# Autodesk Inventor assembly: Weapon Assembly
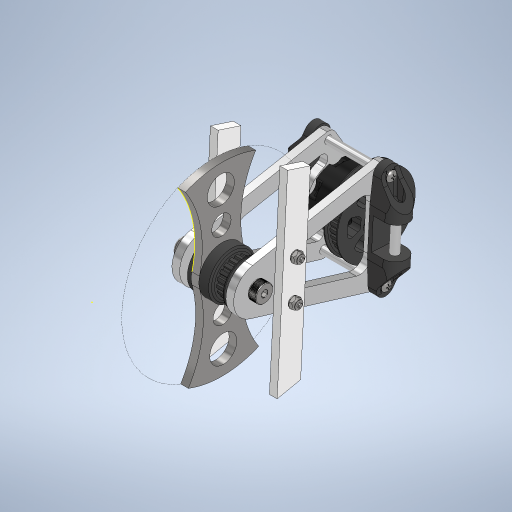
[picture p0: Inventor's stored thumbnail of the model, 512x512]
Saved by Autodesk Inventor 2023.1 (Build 271208000, 208)
## iProperties
Created: 2022-05-21
Part Number: Weapon Assembly
Document SubType Name: Assembly
Designer: Nathan Cai
Mass: 716.023 g
Surface Area: 1380.74 cm^2
Volume: 212.806 cm^3
Density: 3.36467 g/cm^3
Author: Nathan Cai
## Documents named in this file (15)
- E:\Documents\Inventor\0.3rd Lawette - V3.4\Vertical Weapon Assembly (Type A)\Weapon Assembly (Vert A).iam
- E:\Documents\Inventor\0.3rd Lawette - V3.4\Vertical Weapon Assembly (Type A)\Weapon (Weapon-Side Pulley).iam
- E:\Documents\Inventor\0.3rd Lawette - V3.4\Vertical Weapon Assembly (Type A)\90807A139_Same-Size Thread Alloy Steel Shoulder Screw.ipt
- E:\Documents\Inventor\0.3rd Lawette - V3.4\Vertical Weapon Assembly (Type A)\90630A121_High-Strength Steel Nylon-Insert Locknut.ipt
- E:\Documents\Inventor\0.3rd Lawette - V3.4\Vertical Weapon Assembly (Type A)\Weapon (Motor-Side Pulley).iam
- E:\Documents\Inventor\0.3rd Lawette - V3.4\Vertical Weapon Assembly (Type A)\Frame (Clear Side).ipt
- E:\Documents\Inventor\0.3rd Lawette - V3.4\Standoff 1.5in.ipt
- E:\Documents\Inventor\0.3rd Lawette - V3.4\Vertical Weapon Assembly (Type A)\Legs.ipt
- E:\Documents\Inventor\Content Center Files\R2023\en-US\ANSI B18.6.3(27)\ANSI B18.6.3 - 6-32 UNC - 0.75(11).ipt
- E:\Documents\Inventor\Content Center Files\R2023\en-US\SAE J773b\SAE J773b - No. 6. SAE Type L. narrow.ipt
- E:\Documents\Inventor\Content Center Files\R2023\en-US\IFI 100 107(2)\IFI 100_107 - No. 6 - 32 Metal Type.ipt
- E:\Documents\Inventor\0.3rd Lawette - V3.4\Vertical Weapon Assembly (Type A)\Frame (Motor Side).ipt
- E:\Documents\Inventor\0.3rd Lawette - V3.4\Vertical Weapon Assembly (Type A)\Legs_MIR.ipt
- E:\Documents\Inventor\0.3rd Lawette - V3.4\Bracket.ipt
- E:\Documents\Inventor\Content Center Files\R2023\en-US\ANSI B18.6.3(27)\ANSI B18.6.3 - 6-32 UNC - 0.625(11).ipt
## Components (42 placed, 14 different names)
1. Weapon (Weapon-Side Pulley):1 [sub-assembly] — Mate:3
2. Weapon (Motor-Side Pulley):1 [sub-assembly] — Mate:167, Mate:168, Mate:169
3. 90807A139_Same-Size Thread Alloy Steel Shoulder Screw:1 — Mate:1, Mate:2, Mate:3, Mate:9, Mate:10
4. 90630A121_High-Strength Steel Nylon-Insert Locknut:1 — Mate:1, Mate:2
5. Frame (Motor Side):1 — Symmetry:1, Mate:146, Mate:147, Mate:148, Mate:151, Mate:152, Mate:153, Mate:154, Mate:155, Mate:157, Mate:167, Mate:168, Mate:169, Mate:170
6. Frame (Clear Side):1 — Mate:9, Mate:10, Mate:28, Mate:29, Mate:30, Mate:102, Symmetry:1, Mate:159, Mate:160, Mate:161, Mate:162, Mate:163, Mate:165, Mate:173
7. Legs:1 — Mate:28, Mate:29, Mate:30, Mate:164, Mate:166
8. Legs_MIR:1 — Mate:146, Mate:147, Mate:148, Mate:156, Mate:158
9. Bracket:1 — Mate:173, Mate:174, Mate:175, Mate:176, Flush:2, Mate:178, Mate:179, Mate:180, Mate:181, Mate:186, Mate:187, Mate:189, Mate:190
10. Bracket:2 — Mate:170, Mate:171, Mate:172, Mate:177, Flush:1, Mate:182, Mate:183, Mate:184, Mate:185, Mate:188, Mate:192
11. Standoff 1.5in:1 — Mate:102, Mate:171, Mate:174
12. Standoff 1.5in:2 — Mate:172, Mate:175
13. Standoff 1.5in:3 — Mate:176, Flush:2, Mate:191, Mate:193
14. Standoff 1.5in:4 — Mate:177, Flush:1
15. Cross Recessed Truss Head Machine Screw - Type I - Inch No. 6 - 32 - 3/4:8 — Mate:151, Mate:152
16. Conical Spring Washer SAE J773b (Inch) No. 6. SAE Type L. narrow:11 — Mate:155, Mate:156, Insert:21
17. Prevailing Torque Type Hex Nut - Inch (IFI) No. 6 - 32 Metal Type:11 — Insert:21
18. Cross Recessed Truss Head Machine Screw - Type I - Inch No. 6 - 32 - 3/4:10 — Mate:159, Mate:160
19. Conical Spring Washer SAE J773b (Inch) No. 6. SAE Type L. narrow:13 — Mate:163, Mate:164, Insert:23
20. Prevailing Torque Type Hex Nut - Inch (IFI) No. 6 - 32 Metal Type:13 — Insert:23
21. Cross Recessed Truss Head Machine Screw - Type I - Inch No. 6 - 32 - 3/4:14 — Mate:153, Mate:154
22. Conical Spring Washer SAE J773b (Inch) No. 6. SAE Type L. narrow:17 — Mate:157, Mate:158, Insert:22
23. Prevailing Torque Type Hex Nut - Inch (IFI) No. 6 - 32 Metal Type:17 — Insert:22
24. Cross Recessed Truss Head Machine Screw - Type I - Inch No. 6 - 32 - 3/4:15 — Mate:161, Mate:162
25. Conical Spring Washer SAE J773b (Inch) No. 6. SAE Type L. narrow:18 — Mate:165, Mate:166, Insert:24
26. Prevailing Torque Type Hex Nut - Inch (IFI) No. 6 - 32 Metal Type:18 — Insert:24
27. Conical Spring Washer SAE J773b (Inch) No. 6. SAE Type L. narrow:19 — Mate:178, Mate:179, Insert:25
28. Cross Recessed Truss Head Machine Screw - Type I - Inch No. 6 - 32 - 3/4:16 — Insert:25
29. Conical Spring Washer SAE J773b (Inch) No. 6. SAE Type L. narrow:20 — Mate:180, Mate:181, Insert:26
30. Cross Recessed Truss Head Machine Screw - Type I - Inch No. 6 - 32 - 3/4:17 — Insert:26
31. Conical Spring Washer SAE J773b (Inch) No. 6. SAE Type L. narrow:21 — Mate:182, Mate:183, Insert:27
32. Cross Recessed Truss Head Machine Screw - Type I - Inch No. 6 - 32 - 3/4:18 — Insert:27
33. Conical Spring Washer SAE J773b (Inch) No. 6. SAE Type L. narrow:22 — Mate:184, Mate:185, Insert:28
34. Cross Recessed Truss Head Machine Screw - Type I - Inch No. 6 - 32 - 3/4:19 — Insert:28
35. Conical Spring Washer SAE J773b (Inch) No. 6. SAE Type L. narrow:23 — Mate:186, Mate:187, Insert:29
36. Cross Recessed Truss Head Machine Screw - Type I - Inch No. 6 - 32 - 5/8:1 — Insert:29
37. Conical Spring Washer SAE J773b (Inch) No. 6. SAE Type L. narrow:24 — Mate:188, Mate:189, Insert:30
38. Cross Recessed Truss Head Machine Screw - Type I - Inch No. 6 - 32 - 5/8:2 — Insert:30
39. Conical Spring Washer SAE J773b (Inch) No. 6. SAE Type L. narrow:25 — Mate:190, Mate:191, Insert:31
40. Cross Recessed Truss Head Machine Screw - Type I - Inch No. 6 - 32 - 5/8:3 — Insert:31
41. Conical Spring Washer SAE J773b (Inch) No. 6. SAE Type L. narrow:26 — Mate:192, Mate:193, Insert:32
42. Cross Recessed Truss Head Machine Screw - Type I - Inch No. 6 - 32 - 5/8:4 — Insert:32
## Relationships (77: Mate 62, Insert 12, Flush 2, Symmetry 1)
- Mate:1: 90807A139_Same-Size Thread Alloy Steel Shoulder Screw:1 ↔ 90630A121_High-Strength Steel Nylon-Insert Locknut:1
- Mate:2 (50.8 mm): 90807A139_Same-Size Thread Alloy Steel Shoulder Screw:1 ↔ 90630A121_High-Strength Steel Nylon-Insert Locknut:1
- Mate:3: Weapon (Weapon-Side Pulley):1 ↔ 90807A139_Same-Size Thread Alloy Steel Shoulder Screw:1
- [Mate]: 90807A139_Same-Size Thread Alloy Steel Shoulder Screw:1 ↔ Frame (Motor Side):1
- Mate:9: 90807A139_Same-Size Thread Alloy Steel Shoulder Screw:1 ↔ Frame (Clear Side):1
- Mate:10: 90807A139_Same-Size Thread Alloy Steel Shoulder Screw:1 ↔ Frame (Clear Side):1
- [Mate]: Frame (Motor Side):1 ↔ Frame (Clear Side):1
- [Mate]: Frame (Motor Side):1 ↔ Standoff 1.5in:1
- [Mate]: Frame (Motor Side):1 ↔ Standoff 1.5in:2
- [Mate]: Frame (Motor Side):1 ↔ Standoff 1.5in:1
- [Mate]: Frame (Motor Side):1 ↔ Standoff 1.5in:2
- Mate:28: Frame (Clear Side):1 ↔ Legs:1
- Mate:29: Frame (Clear Side):1 ↔ Legs:1
- Mate:30: Frame (Clear Side):1 ↔ Legs:1
- Mate:102: Frame (Clear Side):1 ↔ Standoff 1.5in:1
- [Mate] (0.0254 mm): Weapon (Weapon-Side Pulley):1 ↔ Frame (Motor Side):1
- Symmetry:1: Frame (Motor Side):1 ↔ Frame (Clear Side):1
- Mate:146: Frame (Motor Side):1 ↔ Legs_MIR:1
- Mate:147: Frame (Motor Side):1 ↔ Legs_MIR:1
- Mate:148: Frame (Motor Side):1 ↔ Legs_MIR:1
- Mate:151: Frame (Motor Side):1 ↔ Cross Recessed Truss Head Machine Screw - Type I - Inch No. 6 - 32 - 3/4:8
- Mate:152: Frame (Motor Side):1 ↔ Cross Recessed Truss Head Machine Screw - Type I - Inch No. 6 - 32 - 3/4:8
- Mate:153: Frame (Motor Side):1 ↔ Cross Recessed Truss Head Machine Screw - Type I - Inch No. 6 - 32 - 3/4:14
- Mate:154: Frame (Motor Side):1 ↔ Cross Recessed Truss Head Machine Screw - Type I - Inch No. 6 - 32 - 3/4:14
- Mate:155: Frame (Motor Side):1 ↔ Conical Spring Washer SAE J773b (Inch) No. 6. SAE Type L. narrow:11
- Mate:156: Legs_MIR:1 ↔ Conical Spring Washer SAE J773b (Inch) No. 6. SAE Type L. narrow:11
- Mate:157: Frame (Motor Side):1 ↔ Conical Spring Washer SAE J773b (Inch) No. 6. SAE Type L. narrow:17
- Mate:158: Legs_MIR:1 ↔ Conical Spring Washer SAE J773b (Inch) No. 6. SAE Type L. narrow:17
- Insert:21: Conical Spring Washer SAE J773b (Inch) No. 6. SAE Type L. narrow:11 ↔ Prevailing Torque Type Hex Nut - Inch (IFI) No. 6 - 32 Metal Type:11
- Insert:22: Conical Spring Washer SAE J773b (Inch) No. 6. SAE Type L. narrow:17 ↔ Prevailing Torque Type Hex Nut - Inch (IFI) No. 6 - 32 Metal Type:17
- Mate:159: Frame (Clear Side):1 ↔ Cross Recessed Truss Head Machine Screw - Type I - Inch No. 6 - 32 - 3/4:10
- Mate:160: Frame (Clear Side):1 ↔ Cross Recessed Truss Head Machine Screw - Type I - Inch No. 6 - 32 - 3/4:10
- Mate:161: Frame (Clear Side):1 ↔ Cross Recessed Truss Head Machine Screw - Type I - Inch No. 6 - 32 - 3/4:15
- Mate:162: Frame (Clear Side):1 ↔ Cross Recessed Truss Head Machine Screw - Type I - Inch No. 6 - 32 - 3/4:15
- Mate:163: Frame (Clear Side):1 ↔ Conical Spring Washer SAE J773b (Inch) No. 6. SAE Type L. narrow:13
- Mate:164: Legs:1 ↔ Conical Spring Washer SAE J773b (Inch) No. 6. SAE Type L. narrow:13
- Mate:165: Frame (Clear Side):1 ↔ Conical Spring Washer SAE J773b (Inch) No. 6. SAE Type L. narrow:18
- Mate:166: Legs:1 ↔ Conical Spring Washer SAE J773b (Inch) No. 6. SAE Type L. narrow:18
- Insert:23: Conical Spring Washer SAE J773b (Inch) No. 6. SAE Type L. narrow:13 ↔ Prevailing Torque Type Hex Nut - Inch (IFI) No. 6 - 32 Metal Type:13
- Insert:24: Conical Spring Washer SAE J773b (Inch) No. 6. SAE Type L. narrow:18 ↔ Prevailing Torque Type Hex Nut - Inch (IFI) No. 6 - 32 Metal Type:18
- Mate:167: Weapon (Motor-Side Pulley):1 ↔ Frame (Motor Side):1
- Mate:168: Weapon (Motor-Side Pulley):1 ↔ Frame (Motor Side):1
- Mate:169: Weapon (Motor-Side Pulley):1 ↔ Frame (Motor Side):1
- Mate:170: Frame (Motor Side):1 ↔ Bracket:2
- Mate:171: Bracket:2 ↔ Standoff 1.5in:1
- Mate:172: Bracket:2 ↔ Standoff 1.5in:2
- Mate:173: Frame (Clear Side):1 ↔ Bracket:1
- Mate:174: Bracket:1 ↔ Standoff 1.5in:1
- Mate:175: Bracket:1 ↔ Standoff 1.5in:2
- Mate:176: Bracket:1 ↔ Standoff 1.5in:3
- Mate:177: Bracket:2 ↔ Standoff 1.5in:4
- Flush:1: Bracket:2 ↔ Standoff 1.5in:4
- Flush:2: Bracket:1 ↔ Standoff 1.5in:3
- Mate:178: Bracket:1 ↔ Conical Spring Washer SAE J773b (Inch) No. 6. SAE Type L. narrow:19
- Mate:179: Bracket:1 ↔ Conical Spring Washer SAE J773b (Inch) No. 6. SAE Type L. narrow:19
- Mate:180: Bracket:1 ↔ Conical Spring Washer SAE J773b (Inch) No. 6. SAE Type L. narrow:20
- Mate:181: Bracket:1 ↔ Conical Spring Washer SAE J773b (Inch) No. 6. SAE Type L. narrow:20
- Insert:25: Conical Spring Washer SAE J773b (Inch) No. 6. SAE Type L. narrow:19 ↔ Cross Recessed Truss Head Machine Screw - Type I - Inch No. 6 - 32 - 3/4:16
- Insert:26: Conical Spring Washer SAE J773b (Inch) No. 6. SAE Type L. narrow:20 ↔ Cross Recessed Truss Head Machine Screw - Type I - Inch No. 6 - 32 - 3/4:17
- Mate:182: Bracket:2 ↔ Conical Spring Washer SAE J773b (Inch) No. 6. SAE Type L. narrow:21
- Mate:183: Bracket:2 ↔ Conical Spring Washer SAE J773b (Inch) No. 6. SAE Type L. narrow:21
- Mate:184: Bracket:2 ↔ Conical Spring Washer SAE J773b (Inch) No. 6. SAE Type L. narrow:22
- Mate:185: Bracket:2 ↔ Conical Spring Washer SAE J773b (Inch) No. 6. SAE Type L. narrow:22
- Insert:27: Conical Spring Washer SAE J773b (Inch) No. 6. SAE Type L. narrow:21 ↔ Cross Recessed Truss Head Machine Screw - Type I - Inch No. 6 - 32 - 3/4:18
- Insert:28: Conical Spring Washer SAE J773b (Inch) No. 6. SAE Type L. narrow:22 ↔ Cross Recessed Truss Head Machine Screw - Type I - Inch No. 6 - 32 - 3/4:19
- Mate:186: Bracket:1 ↔ Conical Spring Washer SAE J773b (Inch) No. 6. SAE Type L. narrow:23
- Mate:187: Bracket:1 ↔ Conical Spring Washer SAE J773b (Inch) No. 6. SAE Type L. narrow:23
- Mate:188: Bracket:2 ↔ Conical Spring Washer SAE J773b (Inch) No. 6. SAE Type L. narrow:24
- Mate:189: Bracket:1 ↔ Conical Spring Washer SAE J773b (Inch) No. 6. SAE Type L. narrow:24
- Insert:29: Conical Spring Washer SAE J773b (Inch) No. 6. SAE Type L. narrow:23 ↔ Cross Recessed Truss Head Machine Screw - Type I - Inch No. 6 - 32 - 5/8:1
- Insert:30: Conical Spring Washer SAE J773b (Inch) No. 6. SAE Type L. narrow:24 ↔ Cross Recessed Truss Head Machine Screw - Type I - Inch No. 6 - 32 - 5/8:2
- Mate:190: Bracket:1 ↔ Conical Spring Washer SAE J773b (Inch) No. 6. SAE Type L. narrow:25
- Mate:191: Standoff 1.5in:3 ↔ Conical Spring Washer SAE J773b (Inch) No. 6. SAE Type L. narrow:25
- Mate:192: Bracket:2 ↔ Conical Spring Washer SAE J773b (Inch) No. 6. SAE Type L. narrow:26
- Mate:193: Standoff 1.5in:3 ↔ Conical Spring Washer SAE J773b (Inch) No. 6. SAE Type L. narrow:26
- Insert:31: Conical Spring Washer SAE J773b (Inch) No. 6. SAE Type L. narrow:25 ↔ Cross Recessed Truss Head Machine Screw - Type I - Inch No. 6 - 32 - 5/8:3
- Insert:32: Conical Spring Washer SAE J773b (Inch) No. 6. SAE Type L. narrow:26 ↔ Cross Recessed Truss Head Machine Screw - Type I - Inch No. 6 - 32 - 5/8:4
